# Autodesk Inventor assembly: Level 1
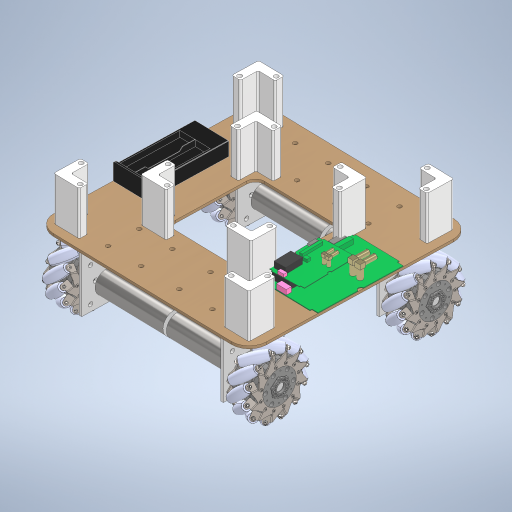
[picture p0: Inventor's stored thumbnail of the model, 512x512]
Saved by Autodesk Inventor 2024 (Build 280153000, 153)
## iProperties
Created: 2023-07-17
Part Number: Level 1
Document SubType Name: Assembly
Designer: javie
Author: javie
## Documents named in this file (8)
- C:\Users\javie\OneDrive\Documents\Inventor\L1\Level 1.iam
- C:\Users\javie\OneDrive\Documents\Inventor\L1\WheelSystem.iam
- C:\Users\javie\OneDrive\Documents\Inventor\L1\Base_Aluminum Plate.ipt
- C:\Users\javie\OneDrive\Documents\Inventor\L1\Metal Braket.ipt
- C:\Users\javie\OneDrive\Documents\Inventor\L1\Base_3D Printed Beam.ipt
- C:\Users\javie\OneDrive\Documents\Inventor\L1\Battery Pack 9.2x4.ipt
- C:\Users\javie\OneDrive\Documents\Inventor\L1\Motor Driver 6.2x4.2 (SCALED).ipt
- C:\Users\javie\OneDrive\Documents\Inventor\L1\Motor Driver 10x4.7 (SCALED).ipt
## Components (20 placed, 7 different names)
1. WheelSystem:1 [sub-assembly] — WS to Bracket 1
2. Base_Aluminum Plate:1 — Braket to Plate_Y1, Braket to Plate_X1, Braket to Plate_Z1, Braket to Plate_Y4, Braket to Plate_X4, Braket to Plate_Z4, Braket to Plate_Y3, Braket to Plate_X3, Braket to Plate_Z3, Braket to Plate_Y2, Braket to Plate_Z2, Braket to Plate_X2, Driver to Plate, Battery to Plate, Insert:5, Insert:6, Insert:7, Insert:8, Insert:9, Insert:10, Insert:11, Insert:12, Insert:13, Insert:14, Insert:15, Insert:16, Insert:17, Insert:18, Insert:19, Insert:20, Flush:9, Flush:10
3. Metal Braket:1 — WS to Bracket 1, Braket to Plate_Y1, Braket to Plate_Z1, Braket to Plate_X1
4. WheelSystem:2 [sub-assembly] — WS to Bracket 2
5. Metal Braket:2 — WS to Bracket 2, Braket to Plate_Y4, Braket to Plate_X4, Braket to Plate_Z4
6. WheelSystem:3 [sub-assembly] — Insert:3
7. Metal Braket:3 — Braket to Plate_Y2, Braket to Plate_Z2, Braket to Plate_X2, WS to Braket 4
8. WheelSystem:4 [sub-assembly] — WS to Braket 4
9. Metal Braket:4 — Braket to Plate_X3, Braket to Plate_Z3, Braket to Plate_Y3, Insert:3
10. Base_3D Printed Beam:1 — Insert:7, Insert:8
11. Base_3D Printed Beam:2 — Insert:11, Insert:12
12. Base_3D Printed Beam:3 — Insert:13, Insert:14
13. Base_3D Printed Beam:4 — Insert:17, Insert:18
14. Battery Pack 9.2x4:1 — Battery to Plate, Flush:9
15. Motor Driver 6.2x4.2 (SCALED):1 — Driver to Driver
16. Motor Driver 10x4.7 (SCALED):1 — Driver to Plate, Driver to Driver, Flush:10
17. Base_3D Printed Beam:5 — Insert:19, Insert:20
18. Base_3D Printed Beam:6 — Insert:9, Insert:10
19. Base_3D Printed Beam:7 — Insert:15, Insert:16
20. Base_3D Printed Beam:8 — Insert:5, Insert:6
## Relationships (37: Insert 20, Flush 10, Mate 7)
- WS to Bracket 1 [Insert]: WheelSystem:1 ↔ Metal Braket:1
- Braket to Plate_Y1 [Mate]: Base_Aluminum Plate:1 ↔ Metal Braket:1
- Braket to Plate_X1 [Flush] (40 mm): Base_Aluminum Plate:1 ↔ Metal Braket:1
- Braket to Plate_Z1 [Flush] (10 mm): Base_Aluminum Plate:1 ↔ Metal Braket:1
- WS to Bracket 2 [Insert]: WheelSystem:2 ↔ Metal Braket:2
- Braket to Plate_Y2 [Mate]: Base_Aluminum Plate:1 ↔ Metal Braket:3
- Braket to Plate_Z2 [Flush] (40 mm): Base_Aluminum Plate:1 ↔ Metal Braket:3
- Braket to Plate_X2 [Flush] (10 mm): Base_Aluminum Plate:1 ↔ Metal Braket:3
- Insert:3: WheelSystem:3 ↔ Metal Braket:4
- Braket to Plate_Y3 [Mate]: Base_Aluminum Plate:1 ↔ Metal Braket:4
- Braket to Plate_X3 [Flush] (10 mm): Base_Aluminum Plate:1 ↔ Metal Braket:4
- Braket to Plate_Z3 [Flush] (40 mm): Base_Aluminum Plate:1 ↔ Metal Braket:4
- WS to Braket 4 [Insert]: Metal Braket:3 ↔ WheelSystem:4
- Braket to Plate_Y4 [Mate]: Base_Aluminum Plate:1 ↔ Metal Braket:2
- Braket to Plate_X4 [Flush] (40 mm): Base_Aluminum Plate:1 ↔ Metal Braket:2
- Braket to Plate_Z4 [Flush] (10 mm): Base_Aluminum Plate:1 ↔ Metal Braket:2
- Driver to Plate [Mate]: Base_Aluminum Plate:1 ↔ Motor Driver 10x4.7 (SCALED):1
- Driver to Driver [Mate]: Motor Driver 6.2x4.2 (SCALED):1 ↔ Motor Driver 10x4.7 (SCALED):1
- Battery to Plate [Mate]: Base_Aluminum Plate:1 ↔ Battery Pack 9.2x4:1
- Insert:5: Base_Aluminum Plate:1 ↔ Base_3D Printed Beam:8
- Insert:6: Base_Aluminum Plate:1 ↔ Base_3D Printed Beam:8
- Insert:7: Base_Aluminum Plate:1 ↔ Base_3D Printed Beam:1
- Insert:8: Base_Aluminum Plate:1 ↔ Base_3D Printed Beam:1
- Insert:9: Base_Aluminum Plate:1 ↔ Base_3D Printed Beam:6
- Insert:10: Base_Aluminum Plate:1 ↔ Base_3D Printed Beam:6
- Insert:11: Base_Aluminum Plate:1 ↔ Base_3D Printed Beam:2
- Insert:12: Base_Aluminum Plate:1 ↔ Base_3D Printed Beam:2
- Insert:13: Base_Aluminum Plate:1 ↔ Base_3D Printed Beam:3
- Insert:14: Base_Aluminum Plate:1 ↔ Base_3D Printed Beam:3
- Insert:15: Base_Aluminum Plate:1 ↔ Base_3D Printed Beam:7
- Insert:16: Base_Aluminum Plate:1 ↔ Base_3D Printed Beam:7
- Insert:17: Base_Aluminum Plate:1 ↔ Base_3D Printed Beam:4
- Insert:18: Base_Aluminum Plate:1 ↔ Base_3D Printed Beam:4
- Insert:19: Base_Aluminum Plate:1 ↔ Base_3D Printed Beam:5
- Insert:20: Base_Aluminum Plate:1 ↔ Base_3D Printed Beam:5
- Flush:9: Base_Aluminum Plate:1 ↔ Battery Pack 9.2x4:1
- Flush:10: Base_Aluminum Plate:1 ↔ Motor Driver 10x4.7 (SCALED):1
## Named parameters: d10_d3 = 0 mm, d11_d3 = 0 mm, d12_d3 = 0 mm
